# Autodesk Inventor assembly: FE-00103
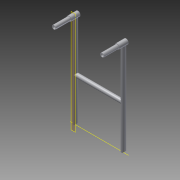
[picture p0: Inventor's stored thumbnail of the model, 180x180]
Saved by Autodesk Inventor 2013 (Build 170138000, 138)
## iProperties
Created: 2013-01-05
Part Number: FE-00103
Document SubType Name: Assembly
Designer: Phillip
_SolveAssemblyDoc: Frame Generator Solve Assembly
_Version: 15.0.0
Author: Phillip
## Documents named in this file (3)
- C:\Users\Moses\Documents\Inventor\2013 Team 3061 Robot\FIRST Arena 2013\Goal Supports\FE-00103.iam
- C:\Users\Moses\Documents\Inventor\2013 Team 3061 Robot\FIRST Arena 2013\Goal Supports\FE-00103Frame.ipt
- C:\Users\Moses\Documents\Inventor\2013 Team 3061 Robot\FIRST Arena 2013\Goal Supports\FE-00103\Frame\Frame0001.iam
## Components (2 placed, 2 different names)
1. FE-00103Frame:1
2. Frame0001:1 [sub-assembly] — Mate:1
## Relationships (1: Mate 1)
- Mate:1: Frame0001:1
